# Autodesk Inventor assembly: shower jig eddie frankenstein
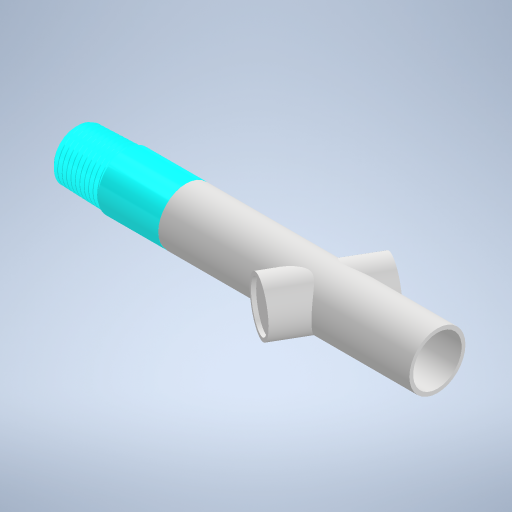
[picture p0: Inventor's stored thumbnail of the model, 512x512]
Saved by Autodesk Inventor 2024.2 (Build 282272000, 272)
## iProperties
Created: 2024-03-20
Part Number: shower jig eddie frankenstein
Document SubType Name: Assembly
Designer: ellix
Author: ellix
## Documents named in this file (3)
- C:\Users\ellix\Documents Local\pipyns.github.io\me\ellie testing\shower jig eddie frankenstein.iam
- C:\Users\ellix\Documents Local\pipyns.github.io\me\ellie testing\eddie church.ipt
- C:\Users\ellix\Documents Local\pipyns.github.io\me\ellie testing\Shower_Jig_-_V3\Shower_Jig_-_V3.ipt
## Components (2 placed, 2 different names)
1. eddie church:1 — Mate:1, Mate:2
2. Shower_Jig_-_V3:1 — Mate:1, Mate:2
## Relationships (2: Mate 2)
- Mate:1: eddie church:1 ↔ Shower_Jig_-_V3:1
- Mate:2: eddie church:1 ↔ Shower_Jig_-_V3:1
